# Autodesk Inventor assembly: Ensamblaje1
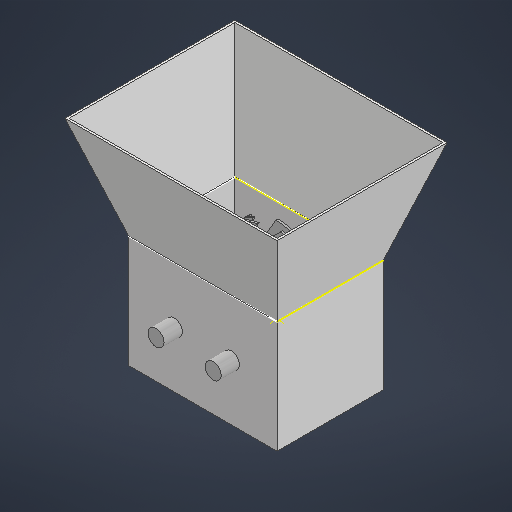
[picture p0: Inventor's stored thumbnail of the model, 512x512]
Saved by Autodesk Inventor 2026.1 (Build 301233020, 233B)
## iProperties
Created: 2025-11-27
Part Number: Ensamblaje1
Document SubType Name: Assembly
Designer: TUF GAMING F15
Author: TUF GAMING F15
## Documents named in this file (6)
- C:\Users\TUF GAMING F15\OneDrive\Escritorio\proyecto SIVAP\Ensamblaje1.iam
- C:\Users\TUF GAMING F15\OneDrive\Escritorio\proyecto SIVAP\eje trituradora pet.ipt
- C:\Users\TUF GAMING F15\OneDrive\Escritorio\proyecto SIVAP\cuchilla molino pet.ipt
- C:\Users\TUF GAMING F15\OneDrive\Escritorio\proyecto SIVAP\espaciador.ipt
- C:\Users\TUF GAMING F15\OneDrive\Escritorio\proyecto SIVAP\tolva.ipt
- C:\Users\TUF GAMING F15\OneDrive\Escritorio\proyecto SIVAP\espaciador1.5mm.ipt
## Components (104 placed, 5 different names)
1. eje trituradora pet:1 — Corredera:1, Corredera:2, Corredera:3, Corredera:4, Corredera:5, Corredera:6, Corredera:7, Corredera:8, Corredera:9, Corredera:10, Corredera:11, Corredera:12, Corredera:13, Corredera:14, Corredera:15, Corredera:16, Corredera:17, Corredera:18, Corredera:19, Corredera:20, Corredera:21, Corredera:22, Corredera:23, Corredera:24, Corredera:25, Corredera:26, Corredera:27, Corredera:28, Corredera:29, Corredera:30, Corredera:31, Corredera:32, Corredera:33, Corredera:34, Corredera:35, Corredera:36, Corredera:37, Corredera:38, Corredera:39, Corredera:40, Corredera:41, Corredera:42, Corredera:43, Corredera:44, Corredera:45, Corredera:46, Corredera:47, Corredera:48, Corredera:49, Corredera:50, De rotación:1
2. espaciador:32 — Corredera:2, Coincidencia:1, Coincidencia:2
3. cuchilla molino pet:1 — Corredera:1, Coincidencia:1, Coincidencia:46
4. cuchilla molino pet:2 — Corredera:4, Coincidencia:3, Coincidencia:4
5. cuchilla molino pet:3 — Corredera:13, Coincidencia:12, Coincidencia:13
6. cuchilla molino pet:4 — Corredera:16, Coincidencia:15, Coincidencia:16
7. cuchilla molino pet:5 — Corredera:22, Coincidencia:21, Coincidencia:22
8. cuchilla molino pet:6 — Corredera:7, Coincidencia:6, Coincidencia:7
9. cuchilla molino pet:7 — Corredera:10, Coincidencia:9, Coincidencia:10
10. cuchilla molino pet:8 — Corredera:19, Coincidencia:18, Coincidencia:19
11. cuchilla molino pet:9 — Corredera:25, Coincidencia:24, Coincidencia:25
12. cuchilla molino pet:10 — Corredera:31, Coincidencia:30, Coincidencia:31
13. espaciador:33 — Corredera:3, Coincidencia:2, Coincidencia:3
14. espaciador:34 — Corredera:5, Coincidencia:4, Coincidencia:5
15. espaciador:35 — Corredera:6, Coincidencia:5, Coincidencia:6
16. espaciador:36 — Corredera:8, Coincidencia:7, Coincidencia:8
17. espaciador:37 — Corredera:9, Coincidencia:8, Coincidencia:9
18. espaciador:38 — Corredera:14, Coincidencia:13, Coincidencia:14
19. espaciador:39 — Corredera:17, Coincidencia:16, Coincidencia:17
20. espaciador:40 — Corredera:20, Coincidencia:19, Coincidencia:20
21. espaciador:41 — Corredera:23, Coincidencia:22, Coincidencia:23
22. espaciador:42 — Corredera:11, Coincidencia:10, Coincidencia:11
23. espaciador:43 — Corredera:12, Coincidencia:11, Coincidencia:12
24. espaciador:44 — Corredera:15, Coincidencia:14, Coincidencia:15
25. espaciador:45 — Corredera:18, Coincidencia:17, Coincidencia:18
26. espaciador:46 — Corredera:21, Coincidencia:20, Coincidencia:21
27. espaciador:47 — Corredera:24, Coincidencia:23, Coincidencia:24
28. espaciador:48 — Corredera:27, Coincidencia:26, Coincidencia:27
29. espaciador:49 — Corredera:30, Coincidencia:29, Coincidencia:30
30. espaciador:50 — Corredera:32, Coincidencia:31, Coincidencia:32
31. espaciador:51 — Corredera:35, Coincidencia:34, Coincidencia:35
32. espaciador:52 — Corredera:36, Coincidencia:35, Coincidencia:36
33. espaciador:53 — Corredera:42, Coincidencia:41, Coincidencia:42
34. espaciador:54 — Corredera:26, Coincidencia:25, Coincidencia:26
35. espaciador:55 — Corredera:29, Coincidencia:28, Coincidencia:29
36. espaciador:56 — Corredera:33, Coincidencia:32, Coincidencia:33
37. espaciador:57 — Corredera:38, Coincidencia:37, Coincidencia:38
38. espaciador:58 — Corredera:39, Coincidencia:38, Coincidencia:39
39. espaciador:59 — Corredera:41, Coincidencia:40, Coincidencia:41
40. cuchilla molino pet:11 — Corredera:34, Coincidencia:33, Coincidencia:34
41. cuchilla molino pet:12 — Corredera:28, Coincidencia:27, Coincidencia:28
42. cuchilla molino pet:13 — Corredera:40, Coincidencia:39, Coincidencia:40
43. cuchilla molino pet:14 — Corredera:43, Coincidencia:42, Coincidencia:43
44. cuchilla molino pet:15 — Corredera:46, Coincidencia:45, Coincidencia:48
45. cuchilla molino pet:16 — Corredera:37, Coincidencia:36, Coincidencia:37
46. espaciador:60 — Corredera:44, Coincidencia:43, Coincidencia:44
47. espaciador:61 — Corredera:45, Coincidencia:44, Coincidencia:45
48. espaciador:62 — Corredera:47, Coincidencia:46, Coincidencia:47
49. espaciador:63 — Corredera:48, Coincidencia:47
50. espaciador:64 — Corredera:49, Coincidencia:48, Coincidencia:49
51. espaciador:65 — Corredera:50, Coincidencia:49, Coincidencia:101
52. tolva:1 — De rotación:1, Nivelación:1, De rotación:2, Coincidencia:101
53. eje trituradora pet:2 — Corredera:51, Coincidencia:50, Corredera:52, Corredera:53, Corredera:54, Corredera:55, Corredera:56, Corredera:57, Corredera:58, Corredera:59, Corredera:60, Corredera:61, Corredera:62, Corredera:63, Corredera:64, Corredera:65, Corredera:66, Corredera:67, Corredera:68, Corredera:69, Corredera:70, Corredera:71, Corredera:72, Corredera:73, Corredera:74, Corredera:75, Corredera:76, Corredera:77, Corredera:78, Corredera:79, Corredera:80, Corredera:81, Corredera:82, Corredera:83, Corredera:84, Corredera:85, Corredera:86, Corredera:87, Corredera:88, Corredera:89, Corredera:90, Corredera:91, Corredera:92, Corredera:93, Corredera:94, Corredera:95, Corredera:96, Corredera:97, Corredera:98, Corredera:99, Corredera:100, Corredera:101, De rotación:2
54. espaciador1.5mm:1 — Corredera:51, Coincidencia:50, Coincidencia:51
55. cuchilla molino pet:17 — Corredera:52, Coincidencia:51, Coincidencia:52
56. cuchilla molino pet:18 — Corredera:61, Coincidencia:60, Coincidencia:61
57. cuchilla molino pet:19 — Corredera:73, Coincidencia:72, Coincidencia:73
58. cuchilla molino pet:20 — Corredera:55, Coincidencia:54, Coincidencia:55
59. cuchilla molino pet:21 — Corredera:64, Coincidencia:63, Coincidencia:64
60. cuchilla molino pet:22 — Corredera:76, Coincidencia:75, Coincidencia:76
61. cuchilla molino pet:23 — Corredera:58, Coincidencia:57, Coincidencia:58
62. cuchilla molino pet:24 — Corredera:67, Coincidencia:66, Coincidencia:67
63. cuchilla molino pet:25 — Corredera:70, Coincidencia:69, Coincidencia:70
64. espaciador:66 — Corredera:53, Coincidencia:52, Coincidencia:53
65. espaciador:67 — Corredera:54, Coincidencia:53, Coincidencia:54
66. espaciador:68 — Corredera:57, Coincidencia:56, Coincidencia:57
67. espaciador:69 — Corredera:56, Coincidencia:55, Coincidencia:56
68. espaciador:70 — Corredera:62, Coincidencia:61, Coincidencia:62
69. espaciador:71 — Corredera:63, Coincidencia:62, Coincidencia:63
70. espaciador:72 — Corredera:65, Coincidencia:64, Coincidencia:65
71. espaciador:73 — Corredera:66, Coincidencia:65, Coincidencia:66
72. espaciador:74 — Corredera:60, Coincidencia:59, Coincidencia:60
73. espaciador:75 — Corredera:59, Coincidencia:58, Coincidencia:59
74. espaciador:76 — Corredera:68, Coincidencia:67, Coincidencia:68
75. espaciador:77 — Corredera:72, Coincidencia:71, Coincidencia:72
76. espaciador:78 — Corredera:74, Coincidencia:73, Coincidencia:74
77. espaciador:79 — Corredera:75, Coincidencia:74, Coincidencia:75
78. espaciador:80 — Corredera:71, Coincidencia:70, Coincidencia:71
79. espaciador:81 — Corredera:69, Coincidencia:68, Coincidencia:69
80. espaciador:82 — Corredera:77, Coincidencia:76, Coincidencia:77
81. espaciador:83 — Corredera:78, Coincidencia:77, Coincidencia:78
82. cuchilla molino pet:26 — Corredera:88, Coincidencia:87, Coincidencia:88
83. cuchilla molino pet:27 — Corredera:79, Coincidencia:78, Coincidencia:79
84. cuchilla molino pet:28 — Corredera:85, Coincidencia:84, Coincidencia:85
85. cuchilla molino pet:29 — Corredera:97, Coincidencia:96, Coincidencia:97
86. cuchilla molino pet:30 — Corredera:100, Coincidencia:99, Coincidencia:100
87. cuchilla molino pet:31 — Corredera:94, Coincidencia:93, Coincidencia:94
88. cuchilla molino pet:32 — Corredera:82, Coincidencia:81, Coincidencia:82
89. cuchilla molino pet:33 — Corredera:91, Coincidencia:90, Coincidencia:91
90. espaciador:84 — Corredera:89, Coincidencia:88, Coincidencia:89
91. espaciador:85 — Corredera:92, Coincidencia:91, Coincidencia:92
92. espaciador:86 — Corredera:87, Coincidencia:86, Coincidencia:87
93. espaciador:87 — Corredera:90, Coincidencia:89, Coincidencia:90
94. espaciador:88 — Corredera:86, Coincidencia:85, Coincidencia:86
95. espaciador:89 — Corredera:93, Coincidencia:92, Coincidencia:93
96. espaciador:90 — Corredera:84, Coincidencia:83, Coincidencia:84
97. espaciador:91 — Corredera:83, Coincidencia:82, Coincidencia:83
98. espaciador:92 — Corredera:81, Coincidencia:80, Coincidencia:81
99. espaciador:93 — Corredera:80, Coincidencia:79, Coincidencia:80
100. espaciador:94 — Corredera:95, Coincidencia:94, Coincidencia:95
101. espaciador:95 — Corredera:96, Coincidencia:95, Coincidencia:96
102. espaciador:96 — Corredera:98, Coincidencia:97, Coincidencia:98
103. espaciador:97 — Corredera:99, Coincidencia:98, Coincidencia:99
104. espaciador1.5mm:2 — Corredera:101, Coincidencia:100
## Relationships (205: TranslationJoint 101, Mate 101, RevoluteJoint 2, Flush 1)
- Corredera:1 [TranslationJoint]: eje trituradora pet:1 ↔ cuchilla molino pet:1
- Corredera:2 [TranslationJoint]: eje trituradora pet:1 ↔ espaciador:32
- Coincidencia:1 [Mate]: espaciador:32 ↔ cuchilla molino pet:1
- Corredera:3 [TranslationJoint]: eje trituradora pet:1 ↔ espaciador:33
- Coincidencia:2 [Mate]: espaciador:32 ↔ espaciador:33
- Corredera:4 [TranslationJoint]: eje trituradora pet:1 ↔ cuchilla molino pet:2
- Coincidencia:3 [Mate]: cuchilla molino pet:2 ↔ espaciador:33
- Corredera:5 [TranslationJoint]: eje trituradora pet:1 ↔ espaciador:34
- Coincidencia:4 [Mate]: cuchilla molino pet:2 ↔ espaciador:34
- Corredera:6 [TranslationJoint]: eje trituradora pet:1 ↔ espaciador:35
- Coincidencia:5 [Mate]: espaciador:34 ↔ espaciador:35
- Corredera:7 [TranslationJoint]: eje trituradora pet:1 ↔ cuchilla molino pet:6
- Coincidencia:6 [Mate]: cuchilla molino pet:6 ↔ espaciador:35
- Corredera:8 [TranslationJoint]: eje trituradora pet:1 ↔ espaciador:36
- Coincidencia:7 [Mate]: cuchilla molino pet:6 ↔ espaciador:36
- Corredera:9 [TranslationJoint]: eje trituradora pet:1 ↔ espaciador:37
- Coincidencia:8 [Mate]: espaciador:36 ↔ espaciador:37
- Corredera:10 [TranslationJoint]: eje trituradora pet:1 ↔ cuchilla molino pet:7
- Coincidencia:9 [Mate]: cuchilla molino pet:7 ↔ espaciador:37
- Corredera:11 [TranslationJoint]: eje trituradora pet:1 ↔ espaciador:42
- Coincidencia:10 [Mate]: cuchilla molino pet:7 ↔ espaciador:42
- Corredera:12 [TranslationJoint]: eje trituradora pet:1 ↔ espaciador:43
- Coincidencia:11 [Mate]: espaciador:42 ↔ espaciador:43
- Corredera:13 [TranslationJoint]: eje trituradora pet:1 ↔ cuchilla molino pet:3
- Coincidencia:12 [Mate]: cuchilla molino pet:3 ↔ espaciador:43
- Corredera:14 [TranslationJoint]: eje trituradora pet:1 ↔ espaciador:38
- Coincidencia:13 [Mate]: cuchilla molino pet:3 ↔ espaciador:38
- Corredera:15 [TranslationJoint]: eje trituradora pet:1 ↔ espaciador:44
- Coincidencia:14 [Mate]: espaciador:38 ↔ espaciador:44
- Corredera:16 [TranslationJoint]: eje trituradora pet:1 ↔ cuchilla molino pet:4
- Coincidencia:15 [Mate]: cuchilla molino pet:4 ↔ espaciador:44
- Corredera:17 [TranslationJoint]: eje trituradora pet:1 ↔ espaciador:39
- Coincidencia:16 [Mate]: cuchilla molino pet:4 ↔ espaciador:39
- Corredera:18 [TranslationJoint]: eje trituradora pet:1 ↔ espaciador:45
- Coincidencia:17 [Mate]: espaciador:39 ↔ espaciador:45
- Corredera:19 [TranslationJoint]: eje trituradora pet:1 ↔ cuchilla molino pet:8
- Coincidencia:18 [Mate]: cuchilla molino pet:8 ↔ espaciador:45
- Corredera:20 [TranslationJoint]: eje trituradora pet:1 ↔ espaciador:40
- Coincidencia:19 [Mate]: cuchilla molino pet:8 ↔ espaciador:40
- Corredera:21 [TranslationJoint]: eje trituradora pet:1 ↔ espaciador:46
- Coincidencia:20 [Mate]: espaciador:40 ↔ espaciador:46
- Corredera:22 [TranslationJoint]: eje trituradora pet:1 ↔ cuchilla molino pet:5
- Coincidencia:21 [Mate]: cuchilla molino pet:5 ↔ espaciador:46
- Corredera:23 [TranslationJoint]: eje trituradora pet:1 ↔ espaciador:41
- Coincidencia:22 [Mate]: cuchilla molino pet:5 ↔ espaciador:41
- Corredera:24 [TranslationJoint]: eje trituradora pet:1 ↔ espaciador:47
- Coincidencia:23 [Mate]: espaciador:41 ↔ espaciador:47
- Corredera:25 [TranslationJoint]: eje trituradora pet:1 ↔ cuchilla molino pet:9
- Coincidencia:24 [Mate]: cuchilla molino pet:9 ↔ espaciador:47
- Corredera:26 [TranslationJoint]: eje trituradora pet:1 ↔ espaciador:54
- Coincidencia:25 [Mate]: cuchilla molino pet:9 ↔ espaciador:54
- Corredera:27 [TranslationJoint]: eje trituradora pet:1 ↔ espaciador:48
- Coincidencia:26 [Mate]: espaciador:48 ↔ espaciador:54
- Corredera:28 [TranslationJoint]: eje trituradora pet:1 ↔ cuchilla molino pet:12
- Coincidencia:27 [Mate]: espaciador:48 ↔ cuchilla molino pet:12
- Corredera:29 [TranslationJoint]: eje trituradora pet:1 ↔ espaciador:55
- Coincidencia:28 [Mate]: espaciador:55 ↔ cuchilla molino pet:12
- Corredera:30 [TranslationJoint]: eje trituradora pet:1 ↔ espaciador:49
- Coincidencia:29 [Mate]: espaciador:49 ↔ espaciador:55
- Corredera:31 [TranslationJoint]: eje trituradora pet:1 ↔ cuchilla molino pet:10
- Coincidencia:30 [Mate]: cuchilla molino pet:10 ↔ espaciador:49
- Corredera:32 [TranslationJoint]: eje trituradora pet:1 ↔ espaciador:50
- Coincidencia:31 [Mate]: cuchilla molino pet:10 ↔ espaciador:50
- Corredera:33 [TranslationJoint]: eje trituradora pet:1 ↔ espaciador:56
- Coincidencia:32 [Mate]: espaciador:50 ↔ espaciador:56
- Corredera:34 [TranslationJoint]: eje trituradora pet:1 ↔ cuchilla molino pet:11
- Coincidencia:33 [Mate]: espaciador:56 ↔ cuchilla molino pet:11
- Corredera:35 [TranslationJoint]: eje trituradora pet:1 ↔ espaciador:51
- Coincidencia:34 [Mate]: espaciador:51 ↔ cuchilla molino pet:11
- Corredera:36 [TranslationJoint]: eje trituradora pet:1 ↔ espaciador:52
- Coincidencia:35 [Mate]: espaciador:51 ↔ espaciador:52
- Corredera:37 [TranslationJoint]: eje trituradora pet:1 ↔ cuchilla molino pet:16
- Coincidencia:36 [Mate]: espaciador:52 ↔ cuchilla molino pet:16
- Corredera:38 [TranslationJoint]: eje trituradora pet:1 ↔ espaciador:57
- Coincidencia:37 [Mate]: espaciador:57 ↔ cuchilla molino pet:16
- Corredera:39 [TranslationJoint]: eje trituradora pet:1 ↔ espaciador:58
- Coincidencia:38 [Mate]: espaciador:57 ↔ espaciador:58
- Corredera:40 [TranslationJoint]: eje trituradora pet:1 ↔ cuchilla molino pet:13
- Coincidencia:39 [Mate]: espaciador:58 ↔ cuchilla molino pet:13
- Corredera:41 [TranslationJoint]: eje trituradora pet:1 ↔ espaciador:59
- Coincidencia:40 [Mate]: espaciador:59 ↔ cuchilla molino pet:13
- Corredera:42 [TranslationJoint]: eje trituradora pet:1 ↔ espaciador:53
- Coincidencia:41 [Mate]: espaciador:53 ↔ espaciador:59
- Corredera:43 [TranslationJoint]: eje trituradora pet:1 ↔ cuchilla molino pet:14
- Coincidencia:42 [Mate]: espaciador:53 ↔ cuchilla molino pet:14
- Corredera:44 [TranslationJoint]: eje trituradora pet:1 ↔ espaciador:60
- Coincidencia:43 [Mate]: cuchilla molino pet:14 ↔ espaciador:60
- Corredera:45 [TranslationJoint]: eje trituradora pet:1 ↔ espaciador:61
- Coincidencia:44 [Mate]: espaciador:60 ↔ espaciador:61
- Corredera:46 [TranslationJoint]: eje trituradora pet:1 ↔ cuchilla molino pet:15
- Coincidencia:45 [Mate]: cuchilla molino pet:15 ↔ espaciador:61
- Corredera:47 [TranslationJoint]: eje trituradora pet:1 ↔ espaciador:62
- Coincidencia:46 [Mate]: cuchilla molino pet:1 ↔ espaciador:62
- Corredera:48 [TranslationJoint]: eje trituradora pet:1 ↔ espaciador:63
- Coincidencia:47 [Mate]: espaciador:62 ↔ espaciador:63
- Corredera:49 [TranslationJoint]: eje trituradora pet:1 ↔ espaciador:64
- Coincidencia:48 [Mate]: cuchilla molino pet:15 ↔ espaciador:64
- Corredera:50 [TranslationJoint]: eje trituradora pet:1 ↔ espaciador:65
- Coincidencia:49 [Mate]: espaciador:64 ↔ espaciador:65
- De rotación:1 [RevoluteJoint] (-30 mm): eje trituradora pet:1 ↔ tolva:1
- Nivelación:1 [Flush] (-150 mm): tolva:1
- Corredera:51 [TranslationJoint]: eje trituradora pet:2 ↔ espaciador1.5mm:1
- Coincidencia:50 [Mate]: eje trituradora pet:2 ↔ espaciador1.5mm:1
- Corredera:52 [TranslationJoint]: eje trituradora pet:2 ↔ cuchilla molino pet:17
- Coincidencia:51 [Mate]: espaciador1.5mm:1 ↔ cuchilla molino pet:17
- Corredera:53 [TranslationJoint]: eje trituradora pet:2 ↔ espaciador:66
- Coincidencia:52 [Mate]: cuchilla molino pet:17 ↔ espaciador:66
- Corredera:54 [TranslationJoint]: eje trituradora pet:2 ↔ espaciador:67
- Coincidencia:53 [Mate]: espaciador:66 ↔ espaciador:67
- Corredera:55 [TranslationJoint]: eje trituradora pet:2 ↔ cuchilla molino pet:20
- Coincidencia:54 [Mate]: cuchilla molino pet:20 ↔ espaciador:67
- Corredera:56 [TranslationJoint]: eje trituradora pet:2 ↔ espaciador:69
- Coincidencia:55 [Mate]: cuchilla molino pet:20 ↔ espaciador:69
- Corredera:57 [TranslationJoint]: eje trituradora pet:2 ↔ espaciador:68
- Coincidencia:56 [Mate]: espaciador:68 ↔ espaciador:69
- Corredera:58 [TranslationJoint]: eje trituradora pet:2 ↔ cuchilla molino pet:23
- Coincidencia:57 [Mate]: cuchilla molino pet:23 ↔ espaciador:68
- Corredera:59 [TranslationJoint]: eje trituradora pet:2 ↔ espaciador:75
- Coincidencia:58 [Mate]: cuchilla molino pet:23 ↔ espaciador:75
- Corredera:60 [TranslationJoint]: eje trituradora pet:2 ↔ espaciador:74
- Coincidencia:59 [Mate]: espaciador:74 ↔ espaciador:75
- Corredera:61 [TranslationJoint]: eje trituradora pet:2 ↔ cuchilla molino pet:18
- Coincidencia:60 [Mate]: cuchilla molino pet:18 ↔ espaciador:74
- Corredera:62 [TranslationJoint]: eje trituradora pet:2 ↔ espaciador:70
- Coincidencia:61 [Mate]: cuchilla molino pet:18 ↔ espaciador:70
- Corredera:63 [TranslationJoint]: eje trituradora pet:2 ↔ espaciador:71
- Coincidencia:62 [Mate]: espaciador:70 ↔ espaciador:71
- Corredera:64 [TranslationJoint]: eje trituradora pet:2 ↔ cuchilla molino pet:21
- Coincidencia:63 [Mate]: cuchilla molino pet:21 ↔ espaciador:71
- Corredera:65 [TranslationJoint]: eje trituradora pet:2 ↔ espaciador:72
- Coincidencia:64 [Mate]: cuchilla molino pet:21 ↔ espaciador:72
- Corredera:66 [TranslationJoint]: eje trituradora pet:2 ↔ espaciador:73
- Coincidencia:65 [Mate]: espaciador:72 ↔ espaciador:73
- Corredera:67 [TranslationJoint]: eje trituradora pet:2 ↔ cuchilla molino pet:24
- Coincidencia:66 [Mate]: cuchilla molino pet:24 ↔ espaciador:73
- Corredera:68 [TranslationJoint]: eje trituradora pet:2 ↔ espaciador:76
- Coincidencia:67 [Mate]: cuchilla molino pet:24 ↔ espaciador:76
- Corredera:69 [TranslationJoint]: eje trituradora pet:2 ↔ espaciador:81
- Coincidencia:68 [Mate]: espaciador:76 ↔ espaciador:81
- Corredera:70 [TranslationJoint]: eje trituradora pet:2 ↔ cuchilla molino pet:25
- Coincidencia:69 [Mate]: cuchilla molino pet:25 ↔ espaciador:81
- Corredera:71 [TranslationJoint]: eje trituradora pet:2 ↔ espaciador:80
- Coincidencia:70 [Mate]: cuchilla molino pet:25 ↔ espaciador:80
- Corredera:72 [TranslationJoint]: eje trituradora pet:2 ↔ espaciador:77
- Coincidencia:71 [Mate]: espaciador:77 ↔ espaciador:80
- Corredera:73 [TranslationJoint]: eje trituradora pet:2 ↔ cuchilla molino pet:19
- Coincidencia:72 [Mate]: cuchilla molino pet:19 ↔ espaciador:77
- Corredera:74 [TranslationJoint]: eje trituradora pet:2 ↔ espaciador:78
- Coincidencia:73 [Mate]: cuchilla molino pet:19 ↔ espaciador:78
- Corredera:75 [TranslationJoint]: eje trituradora pet:2 ↔ espaciador:79
- Coincidencia:74 [Mate]: espaciador:78 ↔ espaciador:79
- Corredera:76 [TranslationJoint]: eje trituradora pet:2 ↔ cuchilla molino pet:22
- Coincidencia:75 [Mate]: cuchilla molino pet:22 ↔ espaciador:79
- Corredera:77 [TranslationJoint]: eje trituradora pet:2 ↔ espaciador:82
- Coincidencia:76 [Mate]: cuchilla molino pet:22 ↔ espaciador:82
- Corredera:78 [TranslationJoint]: eje trituradora pet:2 ↔ espaciador:83
- Coincidencia:77 [Mate]: espaciador:82 ↔ espaciador:83
- Corredera:79 [TranslationJoint]: eje trituradora pet:2 ↔ cuchilla molino pet:27
- Coincidencia:78 [Mate]: espaciador:83 ↔ cuchilla molino pet:27
- Corredera:80 [TranslationJoint]: eje trituradora pet:2 ↔ espaciador:93
- Coincidencia:79 [Mate]: cuchilla molino pet:27 ↔ espaciador:93
- Corredera:81 [TranslationJoint]: eje trituradora pet:2 ↔ espaciador:92
- Coincidencia:80 [Mate]: espaciador:92 ↔ espaciador:93
- Corredera:82 [TranslationJoint]: eje trituradora pet:2 ↔ cuchilla molino pet:32
- Coincidencia:81 [Mate]: cuchilla molino pet:32 ↔ espaciador:92
- Corredera:83 [TranslationJoint]: eje trituradora pet:2 ↔ espaciador:91
- Coincidencia:82 [Mate]: cuchilla molino pet:32 ↔ espaciador:91
- Corredera:84 [TranslationJoint]: eje trituradora pet:2 ↔ espaciador:90
- Coincidencia:83 [Mate]: espaciador:90 ↔ espaciador:91
- Corredera:85 [TranslationJoint]: eje trituradora pet:2 ↔ cuchilla molino pet:28
- Coincidencia:84 [Mate]: cuchilla molino pet:28 ↔ espaciador:90
- Corredera:86 [TranslationJoint]: eje trituradora pet:2 ↔ espaciador:88
- Coincidencia:85 [Mate]: cuchilla molino pet:28 ↔ espaciador:88
- Corredera:87 [TranslationJoint]: eje trituradora pet:2 ↔ espaciador:86
- Coincidencia:86 [Mate]: espaciador:86 ↔ espaciador:88
- Corredera:88 [TranslationJoint]: eje trituradora pet:2 ↔ cuchilla molino pet:26
- Coincidencia:87 [Mate]: cuchilla molino pet:26 ↔ espaciador:86
- Corredera:89 [TranslationJoint]: eje trituradora pet:2 ↔ espaciador:84
- Coincidencia:88 [Mate]: cuchilla molino pet:26 ↔ espaciador:84
- Corredera:90 [TranslationJoint]: eje trituradora pet:2 ↔ espaciador:87
- Coincidencia:89 [Mate]: espaciador:84 ↔ espaciador:87
- Corredera:91 [TranslationJoint]: eje trituradora pet:2 ↔ cuchilla molino pet:33
- Coincidencia:90 [Mate]: cuchilla molino pet:33 ↔ espaciador:87
- Corredera:92 [TranslationJoint]: eje trituradora pet:2 ↔ espaciador:85
- Coincidencia:91 [Mate]: cuchilla molino pet:33 ↔ espaciador:85
- Corredera:93 [TranslationJoint]: eje trituradora pet:2 ↔ espaciador:89
- Coincidencia:92 [Mate]: espaciador:85 ↔ espaciador:89
- Corredera:94 [TranslationJoint]: eje trituradora pet:2 ↔ cuchilla molino pet:31
- Coincidencia:93 [Mate]: cuchilla molino pet:31 ↔ espaciador:89
- Corredera:95 [TranslationJoint]: eje trituradora pet:2 ↔ espaciador:94
- Coincidencia:94 [Mate]: cuchilla molino pet:31 ↔ espaciador:94
- Corredera:96 [TranslationJoint]: eje trituradora pet:2 ↔ espaciador:95
- Coincidencia:95 [Mate]: espaciador:94 ↔ espaciador:95
- Corredera:97 [TranslationJoint]: eje trituradora pet:2 ↔ cuchilla molino pet:29
- Coincidencia:96 [Mate]: cuchilla molino pet:29 ↔ espaciador:95
- Corredera:98 [TranslationJoint]: eje trituradora pet:2 ↔ espaciador:96
- Coincidencia:97 [Mate]: cuchilla molino pet:29 ↔ espaciador:96
- Corredera:99 [TranslationJoint]: eje trituradora pet:2 ↔ espaciador:97
- Coincidencia:98 [Mate]: espaciador:96 ↔ espaciador:97
- Corredera:100 [TranslationJoint]: eje trituradora pet:2 ↔ cuchilla molino pet:30
- Coincidencia:99 [Mate]: cuchilla molino pet:30 ↔ espaciador:97
- Corredera:101 [TranslationJoint]: eje trituradora pet:2 ↔ espaciador1.5mm:2
- Coincidencia:100 [Mate]: cuchilla molino pet:30 ↔ espaciador1.5mm:2
- De rotación:2 [RevoluteJoint] (30 mm): tolva:1 ↔ eje trituradora pet:2
- Coincidencia:101 [Mate]: espaciador:65 ↔ tolva:1
